# Autodesk Inventor assembly: WheelAssembly
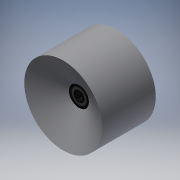
[picture p0: Inventor's stored thumbnail of the model, 180x180]
Saved by Autodesk Inventor 2018 (Build 220112000, 112)
## iProperties
Created: 2019-06-09
Part Number: WheelAssembly
Document SubType Name: Assembly
Designer: anirudh
Author: anirudh
## Documents named in this file (3)
- C:\Users\anirudh\Documents\MARS Fund\Electrical Skateboard\WheelAssembly\WheelAssembly.iam
- C:\Users\anirudh\Documents\MARS Fund\Electrical Skateboard\WheelAssembly\85mmWheel.ipt
- C:\Users\anirudh\Documents\MARS Fund\Electrical Skateboard\WheelAssembly\Skate-Bearing.ipt
## Components (3 placed, 2 different names)
1. 85mmWheel:1 — Mate:1, Mate:3, Mate:4, Mate:5
2. Skate-Bearing:1 — Mate:1, Mate:4
3. Skate-Bearing:2 — Mate:3, Mate:5
## Relationships (4: Mate 4)
- Mate:1: 85mmWheel:1 ↔ Skate-Bearing:1
- Mate:3: 85mmWheel:1 ↔ Skate-Bearing:2
- Mate:4: 85mmWheel:1 ↔ Skate-Bearing:1
- Mate:5: 85mmWheel:1 ↔ Skate-Bearing:2
